# Autodesk Inventor assembly: HTPA23S3M060-A-P10
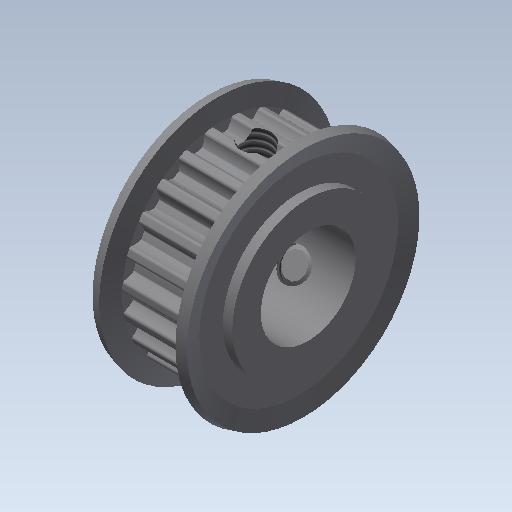
[picture p0: Inventor's stored thumbnail of the model, 512x512]
Saved by Autodesk Inventor 2020.2 (Build 242310000, 310)
## iProperties
Created: 2022-11-04
Part Number: HTPA23S3M060-A-P10
Catalog Web Link: www.cadenas.de
Description: HTPA__S3M060, HTPA__S3M100, HTPA__S3M150, HTPB__S3M060, HTPB__S3M100, HTPB__S3M150, HTPK__S3M060, HTPK__S3M100, HTPK__S3M150, HTPN__S3M060, HTPN__S3M100, HTPN__S3M150, HTPT__S3M060, HTPT__S3M100, HTPT__S3M150, HTPM__S3M060, HTPM__S3M100, HTPM__S3M150, HTPP__S3M060, HTPP__S3M100, HTPP__S3M150, HTPS__S3M060, HTPS__S3M100, KHTPA__S3M060, KHTPA__S3M100, KHTPA__S3M150, KHTPK__S3M060, KHTPK__S3M100, KHTPK__S3M150-High Torque Timing Pulleys S3M Type
Vendor: MISUMI
Document SubType Name: Assembly
Designer: psAdmin
Manufacturer: MISUMI
Mass: 2.68562 g
Surface Area: 25.9941 cm^2
Volume: 2.68562 cm^3
Density: 1 g/cm^3
Category: PARTsolutions
Company: MISUMI
PSOL_IDENT_0: {$CADENAS_DATA/23d-libs/misumi/metric/51_timing_pulleys/htpk_s3m_asmtab.prj},844 {VTYP=3D},{STYP=ASS
PSOL_IDENT_1: TAB},{NB=HTPA23S3M060-A-P10},{LINA=HTPA23S3M060-A-P10},{NN=HTPA__S3M060, HTPA__S3M100, HTPA__S3M150,
PSOL_IDENT_2: HTPB__S3M060, HTPB__S3M100, HTPB__S3M150, HTPK__S3M060, HTPK__S3M100, HTPK__S3M150, HTPN__S3M060, H
PSOL_IDENT_3: TPN__S3M100, HTPN__S3M150, HTPT__S3M060, HTPT__S3M100, HTPT__S3M150, HTPM__S3M060, HTPM__S3M100, HTP
PSOL_IDENT_4: M__S3M150, HTPP__S3M060, HTPP__S3M100, HTPP__S3M150, HTPS__S3M060, HTPS__S3M100, KHTPA__S3M060, KHTP
PSOL_IDENT_5: A__S3M100, KHTPA__S3M150, KHTPK__S3M060, KHTPK__S3M100, KHTPK__S3M150},{DATE=28.10.2022 00:10:07},{G
PSOL_IDENT_6: EOMDATE=15.11.2021 05:07:15},{VERSION=},{LINEID=330},{WBVAR=MATP,ST,TNW,PS,SBS,DD,Z,J,Q,R,S,T,ALT1,A
PSOL_IDENT_7: LT2,M,QSC,QFC,QTC,ALT3,K,KSC,KFC,KTC,ALT4,ZM,ZSC,ZFC,ZTC,ALT5,ALT6,ALT7,FC,ALT8,SRG,ALT9,BTC,TL,ALT1
PSOL_IDENT_8: 0,TPC,ALT11,BC,ALT12,SLH,ALT13,BN},{WBNUMERIC=DD,Z,J,Q,R,S,T,QSC,QFC,QTC,K,KSC,KFC,KTC,ZSC,ZFC,ZTC,F
PSOL_IDENT_9: C,SRG,BTC,TL,BC,SLH,BN}  {NB=HTPA23S3M060-A-P10},{LINA=HTPA23S3M060-A-P10},{KT=DUMMY},{PN=HTPA23S3M0
PSOL_IDENT_10: 60-A-P10},{TYPE=HTPA},{MATP=A2017},{MATPALG='A2017','Aluminum Alloy 2000 series','S45C','1045 Carbon
PSOL_IDENT_11: Steel Equivalent','SUS304','304 Stainless Steel','A6000','6000 Series Aluminum Alloy'},{ST=CA},{STA
PSOL_IDENT_12: LG= 'CA','Clear Anodize','BA','Black Anodize','HAT','Hard Clear Anodize','ENP','Electroless Nickel P
PSOL_IDENT_13: lating' },{NT=23},{TNW=S3M060},{TNWALG= 'S3M060','S3M100','S3M150'    },{BW=6},{PS=A},{PSALG='A','B'
PSOL_IDENT_14: },{SBS=P},{SBSALG= 'H','Round Hole','P','Round Hole + Tap','V','Stepped Hole', 'Y','Both Ends Steppe
PSOL_IDENT_15: d Hole','WB', 'Double Stepped Hole' },{SHSA= 'H','Round Hole','P','Round Hole + Tap','V','Stepped Ho
PSOL_IDENT_16: le', 'Y','Both Ends Stepped Hole','WB', 'Double Stepped Hole' },{SHSB= 'H','Round Hole','P','Round H
PSOL_IDENT_17: ole + Tap','V','Stepped Hole','F','Stepped Hole (Counterbore holes on the boss side)'},{SHSK= '',''
PSOL_IDENT_18: },{SBSPN=-P10},{DD=10.00},{DDALG=[4:4/1],4.5,[5:6/1],6.35,[7:10/1]},{DDHA=[4:4/1],4.5,[5:6/1],6.35,[
PSOL_IDENT_19: 7:12/1]},{DDHBK=0},{DDPA=[4:4/1],4.5,[5:6/1],6.35,[7:10/1]},{DDPBK=0},{DDNA=[8:8/1],[10:11/1]},{DDNB
PSOL_IDENT_20: K=0},{DDNK=0},{DDCA=[10:10/1]},{DDCBK=0},{DDVA=[4:4/1],4.5,[5:6/1],6.35,[7:10/1]},{DDVF=[4:4/1],4.5,
PSOL_IDENT_21: [5:6/1],6.35,[7:8/1]},{DDY=[4:10/1]},{DDWB=[4:8/1]},{Z=0},{ZALG=[0]},{ZQRMIN=12},{ZAMAX=12},{ZBMAX=1
PSOL_IDENT_22: 0},{DDZ=10},{J=0.0},{JALG=[0]},{JMAX=9},{JMIN=2},{JPN=},{QRMAX=12},{QRMIN=12},{WBRMAX=-2.00},{WBQMIN=
PSOL_IDENT_23: 14},{Q=0},{QALG=[0]},{QPN=},{R=0},{RALG=[0]},{S=0.0},{SALG=[0]},{SPN=},{SMAX=5},{T=0.0},{TALG=[0]},{
PSOL_IDENT_24: TPN=},{TMAX=8},{A=7},{W=11},{L=0},{PD=21.96},{OD=21.20},{D=0},{DALG=25},{DE=16},{F=25},{E=16},{BBK=0
PSOL_IDENT_25: .000},{TTK=0.0},{TT=1},{ANG=125.217391},{WL=11},{ALT1=},{ALT1ALG= '','w/o KC90 (Set Screw Angle)','K
PSOL_IDENT_26: C90','with KC90 (Set Screw Angle)' },{ALT1PN=},{ALT2=},{ALT2ALG= '','Not applicable' },{M=N/A},{MALG=
PSOL_IDENT_27: 'N/A' },{MFTALG= 'N/A' },{MSALG= 'N/A' },{M3D=0.000},{KDML=0},{ML=0},{MUL=0},{PITCH=0},{QSC=0.0},{Q
PSOL_IDENT_28: SCALG=0},{QFC=0.0},{QFCALG=0},{QTC=0.0},{QTCALG=0},{QPCDMIN=0},{QPCDMINALG=0},{QPCDMAX=12},{ALT2PN=}
PSOL_IDENT_29: ,{ALT3=},{ALT3ALG= '','Not applicable' },{K=0.0},{KALG=0},{KMIN=4},{KFTMAX=0.0},{KSMAX=0.0},{KSC=0.0
PSOL_IDENT_30: },{KSCALG=0},{KFC=0.0},{KFCALG=0},{KTC=0.0},{KTCALG=0},{KPCDMIN=14},{KPCDMINALG=14},{KPCDMAX=12},{KS
PSOL_IDENT_31: CMIN=14.0},{KSCMINALG=14},{ALT3PN=},{ALT4=},{ALT4ALG= '','Not applicable' },{ALT4MIN=20.5},{ALT4MAX=
PSOL_IDENT_32: 5.5},{ZM=N/A},{ZMALG= 'N/A' },{ZMSALG= 'N/A' },{ZMFTALG= 'N/A' },{ZMDD1=0.0},{ZMDD2=0.0},{ZMHH=0.0},
PSOL_IDENT_33: {ZSC=0.0},{ZSCALG=[0]},{ZFC=0.0},{ZFCALG=[0]},{ZTC=0.0},{ZTCALG=[0]},{ZPCDMIN=0},{ZPCDMINALG=0},{ZPC
PSOL_IDENT_34: DMAX=12},{ALT4PN=},{ALT5=},{ALT5ALG= '','Flange Attached','NFC','with NFC (Flange not Attached)' },{
PSOL_IDENT_35: ALT5PN=},{ALT6=},{ALT6ALG= '','w/o Flange Attached on One Side Only','RFC','with RFC (Flange Attache
PSOL_IDENT_36: d on The Boss Side Only)','LFC','with LFC (Flange Attached on The Opposite Side Only)' },{ALT6PN=},{
PSOL_IDENT_37: ALT7=},{ALT7ALG= '','w/o FC (Flange Cut)','FC','with FC (Flange Cut)' },{FC=0.0},{FCALG=0},{FCMIN=22
PSOL_IDENT_38: .5},{FCMAX=23.0},{ALT7PN=},{ALT8=},{ALT8ALG= '','Not applicable' },{ALT8ALGALG=12},{ALT8DD2=0},{ALT8
PSOL_IDENT_39: MM=0},{ALT8NN=0},{QC=0},{KC=0},{ZC=0},{SRG=0.0},{SRGALG=[0]},{SRGMAX1=0},{SRGMAX=0},{DD2=0.0},{MM=0.
PSOL_IDENT_40: 00},{NN=0.00},{ALT8PN=},{ALT9ALG= '','w/o BTC (Taper for Bearing Holder)','BTC','with BTC (Taper for
PSOL_IDENT_41: Bearing Holder)' },{ALT9=},{BTC9=11},{TL9=1},{BTC=0},{BTCALG=[0]},{TL=0.0},{TLALG=0},{TLMIN=1.0},{T
PSOL_IDENT_42: LMAX=-11.5},{BTCL=0},{BTCD=0},{BTCDALG=16.000},{ALT9PN=},{WLBCTL=11},{ALT10=},{ALT10ALG= '','w/o TPC
PSOL_IDENT_43: (Tapped Hole Dimension)','TPC','with TPC (Tapped Hole Dimension)' },{TPC=N/A},{TPCALG= 'N/A' },{TPC
PSOL_IDENT_44: M=4},{ALT10PN=},{ALT11=},{ALT11ALG= '','Not applicable' },{BC=0.0},{BCALG=0},{BCMIN=7},{BCMAX=-11.5}
PSOL_IDENT_45: ,{BCPLANE=5.5},{M1WBC=5.5},{ALT11PN=},{ALT12=},{ALT12ALG= '','w/o SLH (Set Screw Length)','SLH','wit
PSOL_IDENT_46: h SLH (Set Screw Length)' },{SLH=0},{SLHALG=[0]},{ALT12PN=},{AC=M4x3},{M1=4},{M1L=3},{TAP=0.000},{KY
PSOL_IDENT_47: Y=5},{KTT=5.6},{PLANE=11},{ALT13=},{ALT13ALG= '', 'Not applicable' },{BN=0.0},{BNALG=0},{BNMIN=-10.5
PSOL_IDENT_48: },{BNMAX=-1.0},{ALT13PN=},{PPATH=htpk_s3m/htpa_s3m_asmtpl.prj}
NB: HTPA23S3M060-A-P10
NN: 0
NT: 23
NBSYN: $PN.
LINA: HTPA23S3M060-A-P10
CATALOG: Misumi
PN: HTPA23S3M060-A-P10
MATP: Aluminum Alloy 2000 series
ST: Clear Anodize
TNW: S3M060
BW: 6
PS: A
SBS: Round Hole + Tap
DD: 10
Z: 0
J: 0
Q: 0
R: 0
S: 0
T: 0
A: 7
W: 11
L: 0
PD: 21.96
OD: 21.2
D: 0
F: 25
E: 16
TT: 1
ALT1: w/o KC90 (Set Screw Angle)
ALT2: Not applicable
M: N/A
QSC: 0
QFC: 0
QTC: 0
ALT3: Not applicable
K: 0
KSC: 0
KFC: 0
KTC: 0
ALT4: Not applicable
ZM: N/A
ZMDD1: 0
ZMDD2: 0
ZMHH: 0
ZSC: 0
ZFC: 0
ZTC: 0
ALT5: Flange Attached
ALT6: w/o Flange Attached on One Side Only
ALT7: w/o FC (Flange Cut)
FC: 0
ALT8: Not applicable
SRG: 0
DD2: 0
MM: 0
ALT9: w/o BTC (Taper for Bearing Holder)
BTC: 0
TL: 0
BTCL: 0
BTCD: 0
ALT10: w/o TPC (Tapped Hole Dimension)
TPC: N/A
ALT11: Not applicable
BC: 0
ALT12: w/o SLH (Set Screw Length)
SLH: 0
AC: M4x3
ALT13: Not applicable
BN: 0
SUPPLIER: MISUMI
ARTICLENO: HTPA23S3M060-A-P10
BOMINFO: HTPA23S3M060-A-P10
CREATOR: CADENAS GmbH
Title: HTPA23S3M060-A-P10
Author: Cadenas PARTsolutions
Comments: High Torque Timing Pulleys S3M Type
## Documents named in this file (3)
- C:\Users\Administrator\Documents\kamuy2\Parts\HTPA23S3M060-A-P10_Autodesk_Inventor_2020_20221104\AIS2020\HTPA23S3M060-A-P10.iam
- C:\Users\Administrator\Documents\kamuy2\Parts\HTPA23S3M060-A-P10_Autodesk_Inventor_2020_20221104\AIS2020\HTPA23S3M060-A-P10_b.ipt
- C:\Users\Administrator\Documents\kamuy2\Parts\HTPA23S3M060-A-P10_Autodesk_Inventor_2020_20221104\AIS2020\SET-SCREW4-3.ipt
## Components (3 placed, 2 different names)
1. HTPA23S3M060-A-P10_b:1 — to_screw1_XY@1 <-> CP_XY@2, to_screw1_Z@1 <-> CP_Z@2, to_screw1_YZ@1 <-> CP_YZ@2, to_screw2_XY@1 <-> CP_XY@3, to_screw2_Z@1 <-> CP_Z@3, to_screw2_YZ@1 <-> CP_YZ@3
2. SET-SCREW4-3:1 — to_screw1_XY@1 <-> CP_XY@2, to_screw1_Z@1 <-> CP_Z@2, to_screw1_YZ@1 <-> CP_YZ@2
3. SET-SCREW4-3:2 — to_screw2_XY@1 <-> CP_XY@3, to_screw2_Z@1 <-> CP_Z@3, to_screw2_YZ@1 <-> CP_YZ@3
## Relationships (6: Mate 4, Angle 2)
- to_screw1_XY@1 <-> CP_XY@2 [Mate]: HTPA23S3M060-A-P10_b:1 ↔ SET-SCREW4-3:1
- to_screw1_Z@1 <-> CP_Z@2 [Mate]: HTPA23S3M060-A-P10_b:1 ↔ SET-SCREW4-3:1
- to_screw1_YZ@1 <-> CP_YZ@2 [Angle] (0 deg): HTPA23S3M060-A-P10_b:1 ↔ SET-SCREW4-3:1
- to_screw2_XY@1 <-> CP_XY@3 [Mate]: HTPA23S3M060-A-P10_b:1 ↔ SET-SCREW4-3:2
- to_screw2_Z@1 <-> CP_Z@3 [Mate]: HTPA23S3M060-A-P10_b:1 ↔ SET-SCREW4-3:2
- to_screw2_YZ@1 <-> CP_YZ@3 [Angle] (0 deg): HTPA23S3M060-A-P10_b:1 ↔ SET-SCREW4-3:2
